# Autodesk Inventor assembly: TS-103-T-A
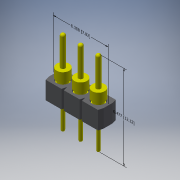
[picture p0: Inventor's stored thumbnail of the model, 180x180]
Saved by Autodesk Inventor 2019 (Build 230136000, 136)
## iProperties
Category: PARTsolutions
Company: SAMTEC
Created: 2024-02-02
Part Number: TS-103-T-A
Catalog Web Link: www.cadenas.de
Description: TS Series-TS Series - (2,54 mm) .100'' Precision Machined Terminal Strips
Vendor: SAMTEC
Document SubType Name: Assembly
Designer: psAdmin
Manufacturer: SAMTEC
Mass: 0.0624283 g
Surface Area: 2.38091 cm^2
Volume: 0.0624283 cm^3
Density: 1 g/cm^3
Title: TS-103-T-A
Author: Cadenas PARTsolutions
Comments: TS Series - (2,54 mm) .100'' Precision Machined Terminal Strips
PSOL_IDENT_0: {$CADENAS_DATA/23d-libs/samtec/modelling/ts/ts_asmtab.prj},189 {VTYP=3D},{STYP=ASSTAB},{NB=TS-103-T-
PSOL_IDENT_1: A},{LINA=TS-103-T-A},{NN=TS Series},{DATE=04.03.2020 14:26:01},{GEOMDATE=03.03.2020 07:44:07},{VERSI
PSOL_IDENT_2: ON=},{LINEID=10},{WBVAR=POS,PLOPT,LS},{WBNUMERIC=}  {NB=TS-103-T-A},{LINA=TS-103-T-A},{KT=DUMMY},{PN=
PSOL_IDENT_3: TS-103-T-A},{SERIES=TS},{ROW=TS},{POS=03},{POSN=3},{POSALG=  '01','-01','02','-02','03','-03','04','
PSOL_IDENT_4: -04','05','-05','06','-06','07','-07','08','-08','09','-09','10','-10','11','-11','12','-12','13','-
PSOL_IDENT_5: 13','14','-14','15','-15','16','-16','17','-17','18','-18','19','-19','20','-20','21','-21','22','-2
PSOL_IDENT_6: 2','23','-23','24','-24','25','-25','26','-26','27','-27','28','-28','29','-29','30','-30','31','-31'
PSOL_IDENT_7: ,'32','-32' },{POSPN=03},{PLOPT=T},{PLOPTALG= 'G','-G: 20µ\" Selective Gold','T','-T: Matte Tin' },{
PSOL_IDENT_8: LS=A},{LSALG= 'AA','-AA','A','-A','A-1','-A-1','A-2','-A-2','C','-C','C-1','-C-1','C-2','-C-2','G-1'
PSOL_IDENT_9: ,'-G-1','J','-J','L-1','-L-1','L-2','-L-2','L-3','-L-3','B','Non-standard option - Please contact SA
PSOL_IDENT_10: MTEC: -B','B-2','Non-standard option - Please contact SAMTEC: -B-2','E','Non-standard option - Pleas
PSOL_IDENT_11: e contact SAMTEC: -E','K','Non-standard option - Please contact SAMTEC: -K','N','Non-standard option
PSOL_IDENT_12: - Please contact SAMTEC: -N','Q-3','Non-standard option - Please contact SAMTEC: -Q-3' },{A=0.100},
PSOL_IDENT_13: {B=0.10000},{C=0.143},{D=0.018},{D2=0.018},{E=0.156},{F=0.166},{G=0.008},{H=0.070},{I=0.052},{J=0.05
PSOL_IDENT_14: 2},{PL=0.477},{SQ=0.000},{W=0.30000},{FIG=2},{X=0},{PPATH=parts/ts_asmtpl.prj}
NB: TS-103-T-A
NN: TS Series
NT: TS Series - (2,54 mm) .100'' Precision Machined Terminal Strips
NBSYN: $PN.
LINA: TS-103-T-A
CATALOG: Samtec
PN: TS-103-T-A
SERIES: TS
POS: -03
PLOPT: -T: Matte Tin
LS: -A
SUPPLIER: SAMTEC
ARTICLENO: TS-103-T-A
BOMINFO: TS-103-T-A
CREATOR: CADENAS GmbH
## Documents named in this file (3)
- e:\temp\worker_COMMON_2\temp\tmp_5540_12_Rc8ir\format_0\TS-103-T-A.iam
- e:\temp\worker_COMMON_2\temp\tmp_5540_12_Rc8ir\format_0\TS-103-G-A_socket.ipt
- e:\temp\worker_COMMON_2\temp\tmp_5540_12_Rc8ir\format_0\-101-G-A_pins.ipt
## Components (4 placed, 2 different names)
1. TS-103-G-A_socket:1 — to_pin_1_XY@1 <-> pins_XY@2, to_pin_1_Z@1 <-> pins_Z@2, to_pin_1_YZ@1 <-> pins_YZ@2, to_pin_2_XY@1 <-> pins_XY@3, to_pin_2_Z@1 <-> pins_Z@3, to_pin_2_YZ@1 <-> pins_YZ@3, to_pin_3_XY@1 <-> pins_XY@4, to_pin_3_Z@1 <-> pins_Z@4, to_pin_3_YZ@1 <-> pins_YZ@4
2. -101-G-A_pins:1 — to_pin_1_XY@1 <-> pins_XY@2, to_pin_1_Z@1 <-> pins_Z@2, to_pin_1_YZ@1 <-> pins_YZ@2
3. -101-G-A_pins:2 — to_pin_2_XY@1 <-> pins_XY@3, to_pin_2_Z@1 <-> pins_Z@3, to_pin_2_YZ@1 <-> pins_YZ@3
4. -101-G-A_pins:3 — to_pin_3_XY@1 <-> pins_XY@4, to_pin_3_Z@1 <-> pins_Z@4, to_pin_3_YZ@1 <-> pins_YZ@4
## Relationships (9: Flush 3, Mate 3, Angle 3)
- to_pin_1_XY@1 <-> pins_XY@2 [Flush]: TS-103-G-A_socket:1 ↔ -101-G-A_pins:1
- to_pin_1_Z@1 <-> pins_Z@2 [Mate]: TS-103-G-A_socket:1 ↔ -101-G-A_pins:1
- to_pin_1_YZ@1 <-> pins_YZ@2 [Angle] (0 deg): TS-103-G-A_socket:1 ↔ -101-G-A_pins:1
- to_pin_2_XY@1 <-> pins_XY@3 [Flush]: TS-103-G-A_socket:1 ↔ -101-G-A_pins:2
- to_pin_2_Z@1 <-> pins_Z@3 [Mate]: TS-103-G-A_socket:1 ↔ -101-G-A_pins:2
- to_pin_2_YZ@1 <-> pins_YZ@3 [Angle] (0 deg): TS-103-G-A_socket:1 ↔ -101-G-A_pins:2
- to_pin_3_XY@1 <-> pins_XY@4 [Flush]: TS-103-G-A_socket:1 ↔ -101-G-A_pins:3
- to_pin_3_Z@1 <-> pins_Z@4 [Mate]: TS-103-G-A_socket:1 ↔ -101-G-A_pins:3
- to_pin_3_YZ@1 <-> pins_YZ@4 [Angle] (0 deg): TS-103-G-A_socket:1 ↔ -101-G-A_pins:3
